# Autodesk Inventor assembly: pickGuardAssembly01
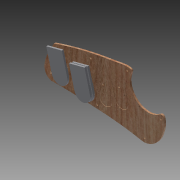
[picture p0: Inventor's stored thumbnail of the model, 180x180]
Saved by Autodesk Inventor 2013 (Build 170138000, 138)
## iProperties
Created: 2014-04-23
Part Number: pickGuardAssembly01
Document SubType Name: Assembly
Designer: Nano
Author: Nano
## Documents named in this file (3)
- C:\Users\Nano\Documents\InventorByron\InventorMasterProject\gyroPhone01\pickGuardAssembly01.iam
- C:\Users\Nano\Documents\InventorByron\InventorMasterProject\gyroPhone01\pickGuard03.ipt
- C:\Users\Nano\Documents\InventorByron\InventorMasterProject\gyroPhone01\fingerBase01.ipt
## Components (4 placed, 2 different names)
1. pickGuard03:1 — Flush:1, Flush:2
2. fingerBase01:1 — Flush:1, Flush:2
3. fingerBase01:2
4. fingerBase01:3
## Relationships (2: Flush 2)
- Flush:1: pickGuard03:1 ↔ fingerBase01:1
- Flush:2: pickGuard03:1 ↔ fingerBase01:1
